# Autodesk Inventor assembly: Collector wheel
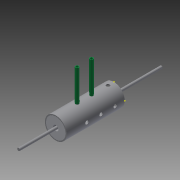
[picture p0: Inventor's stored thumbnail of the model, 180x180]
Saved by Autodesk Inventor 2015 (Build 190159000, 159)
## iProperties
Created: 2014-11-17
Part Number: Collector wheel
Document SubType Name: Assembly
Designer: lethcoec
Author: lethcoec
## Documents named in this file (3)
- \\st-svr\studenthdrives$\18\LethcoeC\FTC Cascade effect\Collector wheel.iam
- \\st-svr\studenthdrives$\18\LethcoeC\FTC Cascade effect\collector.ipt
- \\st-svr\studenthdrives$\18\LethcoeC\FTC Cascade effect\Imported Components\Axle250mm\Axle250mm.ipt
## Components (2 placed, 2 different names)
1. collector:1 — Mate:1
2. Axle250mm:1 — Mate:1
## Relationships (1: Mate 1)
- Mate:1: collector:1 ↔ Axle250mm:1
